# Autodesk Inventor assembly: Servo-Bracket Assembly
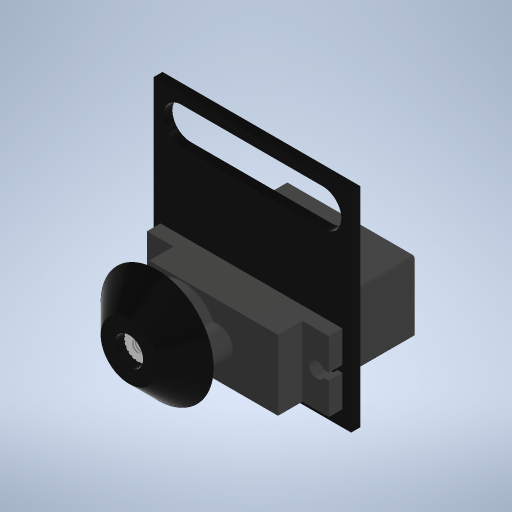
[picture p0: Inventor's stored thumbnail of the model, 512x512]
Saved by Autodesk Inventor 2023 (Build 270158000, 158)
## iProperties
Created: 2022-10-04
Part Number: Servo-Bracket Assembly
Document SubType Name: Assembly
Designer: Raker
Author: Raker
## Documents named in this file (4)
- D:\College Stuff\ATMAE Robotics\Pill Dispenser Robot\Plates and Brackets\Servo-Bracket Assembly.iam
- D:\College Stuff\ATMAE Robotics\Pill Dispenser Robot\Plates and Brackets\Servo_mount_flat.ipt
- D:\College Stuff\ATMAE Robotics\Pill Dispenser Robot\Electronics\Servos\MG90S Servo Motor.ipt
- D:\College Stuff\ATMAE Robotics\Pill Dispenser Robot\Servo Parts and Assemblies\Servo Wheel.ipt
## Components (3 placed, 3 different names)
1. Servo_mount_flat:1 — Mate:1, Mate:2, Mate:3
2. MG90S Servo Motor:1 — Mate:1, Mate:2, Mate:3, Mate:4, Mate:5, Angle:1
3. Servo Wheel:1 — Mate:4, Mate:5, Angle:1
## Relationships (6: Mate 5, Angle 1)
- Mate:1: Servo_mount_flat:1 ↔ MG90S Servo Motor:1
- Mate:2: Servo_mount_flat:1 ↔ MG90S Servo Motor:1
- Mate:3: Servo_mount_flat:1 ↔ MG90S Servo Motor:1
- Mate:4: MG90S Servo Motor:1 ↔ Servo Wheel:1
- Mate:5: MG90S Servo Motor:1 ↔ Servo Wheel:1
- Angle:1 (180 deg): MG90S Servo Motor:1 ↔ Servo Wheel:1
